# Autodesk Inventor assembly: Subensamble estaciones
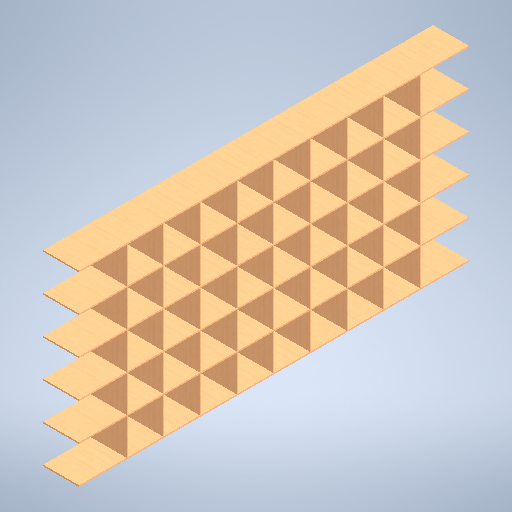
[picture p0: Inventor's stored thumbnail of the model, 512x512]
Saved by Autodesk Inventor 2025.2 (Build 292293000, 293)
## iProperties
Created: 2025-05-13
Part Number: Subensamble estaciones
Document SubType Name: Assembly
Designer: USER
Author: USER
## Documents named in this file (4)
- C:\Users\USER\Desktop\TESIS\STORAGE_FINAL\Subensamble estaciones.iam
- C:\Users\USER\Desktop\TESIS\STORAGE_FINAL\Base.ipt
- C:\Users\USER\Desktop\TESIS\STORAGE_FINAL\Separador.ipt
- C:\Users\USER\Desktop\TESIS\STORAGE_FINAL\Base_Entera.ipt
## Components (15 placed, 3 different names)
1. Base:2 — Mate:34, Mate:35, Mate:36, Flush:3
2. Base:3 — Mate:31, Mate:32, Mate:33
3. Base:4 — Mate:28, Mate:29, Mate:30
4. Base:5 — Mate:1, Mate:2, Mate:3, Mate:4, Mate:5, Mate:6, Mate:7, Mate:8, Mate:9, Mate:10, Mate:11, Mate:12, Mate:13, Mate:14, Mate:15, Mate:16, Mate:17, Mate:18, Mate:19, Mate:20, Mate:21, Mate:22, Mate:23, Mate:24, Mate:25, Mate:26, Mate:27, Flush:1
5. Separador:1 — Mate:1, Mate:2, Mate:7, Mate:28, Mate:29, Mate:30, Mate:31, Mate:32, Mate:33, Mate:34, Mate:35, Mate:36
6. Separador:2 — Mate:5, Mate:6, Mate:9
7. Separador:3 — Mate:10, Mate:11, Mate:12
8. Separador:4 — Mate:13, Mate:14, Mate:15
9. Separador:5 — Mate:16, Mate:17, Mate:18
10. Separador:6 — Mate:19, Mate:20, Mate:21, Mate:37
11. Separador:7 — Mate:22, Mate:23, Mate:24
12. Separador:8 — Mate:25, Mate:26, Mate:27, Flush:2, Mate:39, Flush:4
13. Separador:9 — Mate:3, Mate:4, Mate:8
14. Base_Entera:1 — Mate:37, Flush:1, Flush:2
15. Base_Entera:2 — Flush:3, Mate:39, Flush:4
## Relationships (42: Mate 38, Flush 4)
- Mate:1: Base:5 ↔ Separador:1
- Mate:2: Base:5 ↔ Separador:1
- Mate:3: Base:5 ↔ Separador:9
- Mate:4: Base:5 ↔ Separador:9
- Mate:5: Base:5 ↔ Separador:2
- Mate:6: Base:5 ↔ Separador:2
- Mate:7: Base:5 ↔ Separador:1
- Mate:8: Base:5 ↔ Separador:9
- Mate:9: Base:5 ↔ Separador:2
- Mate:10: Base:5 ↔ Separador:3
- Mate:11: Base:5 ↔ Separador:3
- Mate:12: Base:5 ↔ Separador:3
- Mate:13: Base:5 ↔ Separador:4
- Mate:14: Base:5 ↔ Separador:4
- Mate:15: Base:5 ↔ Separador:4
- Mate:16: Base:5 ↔ Separador:5
- Mate:17: Base:5 ↔ Separador:5
- Mate:18: Base:5 ↔ Separador:5
- Mate:19: Base:5 ↔ Separador:6
- Mate:20: Base:5 ↔ Separador:6
- Mate:21: Base:5 ↔ Separador:6
- Mate:22: Base:5 ↔ Separador:7
- Mate:23: Base:5 ↔ Separador:7
- Mate:24: Base:5 ↔ Separador:7
- Mate:25: Base:5 ↔ Separador:8
- Mate:26: Base:5 ↔ Separador:8
- Mate:27: Base:5 ↔ Separador:8
- Mate:28: Base:4 ↔ Separador:1
- Mate:29: Base:4 ↔ Separador:1
- Mate:30: Base:4 ↔ Separador:1
- Mate:31: Base:3 ↔ Separador:1
- Mate:32: Base:3 ↔ Separador:1
- Mate:33: Base:3 ↔ Separador:1
- Mate:34: Base:2 ↔ Separador:1
- Mate:35: Base:2 ↔ Separador:1
- Mate:36: Base:2 ↔ Separador:1
- Mate:37: Separador:6 ↔ Base_Entera:1
- Flush:1: Base:5 ↔ Base_Entera:1
- Flush:2: Separador:8 ↔ Base_Entera:1
- Flush:3: Base:2 ↔ Base_Entera:2
- Mate:39: Separador:8 ↔ Base_Entera:2
- Flush:4: Separador:8 ↔ Base_Entera:2
